# Autodesk Inventor assembly: Assembly1
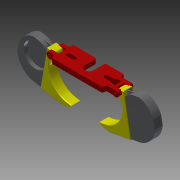
[picture p0: Inventor's stored thumbnail of the model, 180x180]
Saved by Autodesk Inventor 2014 (Build 180170000, 170)
## iProperties
Created: 2016-11-16
Part Number: Assembly1
Document SubType Name: Assembly
Designer: Rubén
Author: Rubén
## Documents named in this file (4)
- C:\Users\Rubén\Dropbox\Proyectos\Puma-printer\Piezas Prusa i3 Steel\Cooler\Assembly1.iam
- C:\Users\Rubén\Dropbox\Proyectos\Puma-printer\Piezas Prusa i3 Steel\Cooler\6mm_groove_mounting_plate.ipt
- C:\Users\Rubén\Dropbox\Proyectos\Puma-printer\Piezas Prusa i3 Steel\Cooler\Blower duct.ipt
- C:\Users\Rubén\Dropbox\Proyectos\Puma-printer\Piezas Prusa i3 Steel\Cooler\Blower.ipt
## Components (5 placed, 3 different names)
1. 6mm_groove_mounting_plate:1 — Mate:4, Mate:5, Mate:6, Mate:7, Angle:1, Angle:2
2. Blower duct:1 — Mate:6, Mate:7, Mate:8, Mate:9, Mate:10, Angle:1
3. Blower duct:2 — Mate:1, Mate:2, Mate:3, Mate:4, Mate:5, Angle:2
4. Blower:1 — Mate:8, Mate:9, Mate:10
5. Blower:2 — Mate:1, Mate:2, Mate:3
## Relationships (12: Mate 10, Angle 2)
- Mate:1: Blower duct:2 ↔ Blower:2
- Mate:2: Blower duct:2 ↔ Blower:2
- Mate:3: Blower duct:2 ↔ Blower:2
- Mate:4: 6mm_groove_mounting_plate:1 ↔ Blower duct:2
- Mate:5: 6mm_groove_mounting_plate:1 ↔ Blower duct:2
- Mate:6: 6mm_groove_mounting_plate:1 ↔ Blower duct:1
- Mate:7: 6mm_groove_mounting_plate:1 ↔ Blower duct:1
- Mate:8: Blower duct:1 ↔ Blower:1
- Mate:9: Blower duct:1 ↔ Blower:1
- Mate:10: Blower duct:1 ↔ Blower:1
- Angle:1 (-80 deg): 6mm_groove_mounting_plate:1 ↔ Blower duct:1
- Angle:2 (80 deg): 6mm_groove_mounting_plate:1 ↔ Blower duct:2
